# Autodesk Inventor assembly: full_layout_test
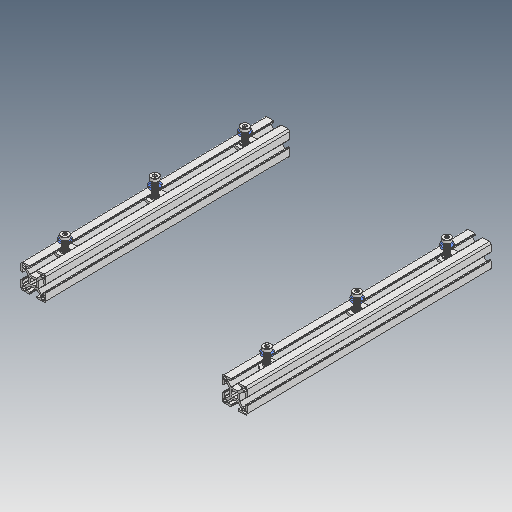
[picture p0: Inventor's stored thumbnail of the model, 512x512]
Saved by Autodesk Inventor 2025.4 (Build 294407020, 407B)
## iProperties
Created: 2026-09-08
Part Number: full_layout_test
Document SubType Name: Assembly
Designer: Aiden
Author: Aiden
## Documents named in this file (7)
- C:\Users\Aiden\Documents\GitHub\coldex-instrumentation\3d_models\mounting_hardware\dummy_parts\full_layout_test.iam
- C:\Users\Aiden\Documents\GitHub\coldex-instrumentation\3d_models\mounting_hardware\dummy_parts\acrylic_base.ipt
- C:\Users\Aiden\Documents\GitHub\coldex-instrumentation\3d_models\mounting_hardware\dummy_parts\acrylic_cover.ipt
- C:\Users\Aiden\Documents\GitHub\coldex-instrumentation\3d_models\mounting_hardware\McMaster\30mm_1ft_T-Slotted Framing.ipt
- C:\Users\Aiden\Documents\GitHub\coldex-instrumentation\3d_models\mounting_hardware\McMaster\30mm_teenut_T-Slotted Framing.ipt
- C:\Users\Aiden\Documents\GitHub\coldex-instrumentation\3d_models\mounting_hardware\McMaster\0.257in_innerD_Moisture-Resistant Cushioning Washer.ipt
- C:\Users\Aiden\Documents\GitHub\coldex-instrumentation\3d_models\mounting_hardware\McMaster\m6_18mm_18-8 Stainless Steel Low-Profile Socket Head Screws.ipt
## Components (22 placed, 6 different names)
1. acrylic_base:1 — Flush:1, Flush:2, Mate:1, Mate:2, Flush:3, Flush:4, Mate:9, Mate:10, Mate:11, Mate:12, Mate:13, Mate:14, Mate:21, Mate:22, Mate:23, Mate:24, Mate:25, Mate:26
2. acrylic_cover:1 — Flush:1, Flush:2
3. 30mm_1ft_T-Slotted Framing:1 — Mate:1, Flush:4, Mate:3, Mate:4, Mate:5, Tangent:2
4. 30mm_1ft_T-Slotted Framing:2 — Mate:2, Flush:3, Mate:6, Mate:7, Mate:8, Tangent:1
5. 30mm_teenut_T-Slotted Framing:1 — Mate:5, Mate:9
6. 30mm_teenut_T-Slotted Framing:2 — Mate:3, Mate:10
7. 30mm_teenut_T-Slotted Framing:3 — Mate:4, Mate:11, Tangent:2
8. 30mm_teenut_T-Slotted Framing:4 — Mate:7, Mate:13
9. 30mm_teenut_T-Slotted Framing:5 — Mate:6, Mate:14
10. 30mm_teenut_T-Slotted Framing:6 — Mate:8, Mate:12, Tangent:1
11. m6_18mm_18-8 Stainless Steel Low-Profile Socket Head Screws:1
12. m6_18mm_18-8 Stainless Steel Low-Profile Socket Head Screws:2
13. m6_18mm_18-8 Stainless Steel Low-Profile Socket Head Screws:3
14. m6_18mm_18-8 Stainless Steel Low-Profile Socket Head Screws:4
15. m6_18mm_18-8 Stainless Steel Low-Profile Socket Head Screws:5
16. m6_18mm_18-8 Stainless Steel Low-Profile Socket Head Screws:6
17. 0.257in_innerD_Moisture-Resistant Cushioning Washer:1 — Mate:22
18. 0.257in_innerD_Moisture-Resistant Cushioning Washer:2 — Mate:23
19. 0.257in_innerD_Moisture-Resistant Cushioning Washer:3 — Mate:24
20. 0.257in_innerD_Moisture-Resistant Cushioning Washer:4 — Mate:26
21. 0.257in_innerD_Moisture-Resistant Cushioning Washer:5 — Mate:25
22. 0.257in_innerD_Moisture-Resistant Cushioning Washer:6 — Mate:21
## Relationships (39: Mate 33, Flush 4, Tangent 2)
- Flush:1: acrylic_base:1 ↔ acrylic_cover:1
- Flush:2: acrylic_base:1 ↔ acrylic_cover:1
- Mate:1: acrylic_base:1 ↔ 30mm_1ft_T-Slotted Framing:1
- Mate:2: acrylic_base:1 ↔ 30mm_1ft_T-Slotted Framing:2
- Flush:3: acrylic_base:1 ↔ 30mm_1ft_T-Slotted Framing:2
- Flush:4: acrylic_base:1 ↔ 30mm_1ft_T-Slotted Framing:1
- Mate:3: 30mm_1ft_T-Slotted Framing:1 ↔ 30mm_teenut_T-Slotted Framing:2
- Mate:4: 30mm_1ft_T-Slotted Framing:1 ↔ 30mm_teenut_T-Slotted Framing:3
- Mate:5: 30mm_1ft_T-Slotted Framing:1 ↔ 30mm_teenut_T-Slotted Framing:1
- Mate:6: 30mm_1ft_T-Slotted Framing:2 ↔ 30mm_teenut_T-Slotted Framing:5
- Mate:7: 30mm_1ft_T-Slotted Framing:2 ↔ 30mm_teenut_T-Slotted Framing:4
- Mate:8: 30mm_1ft_T-Slotted Framing:2 ↔ 30mm_teenut_T-Slotted Framing:6
- Mate:9: acrylic_base:1 ↔ 30mm_teenut_T-Slotted Framing:1
- Mate:10: acrylic_base:1 ↔ 30mm_teenut_T-Slotted Framing:2
- Mate:11: acrylic_base:1 ↔ 30mm_teenut_T-Slotted Framing:3
- Mate:12: acrylic_base:1 ↔ 30mm_teenut_T-Slotted Framing:6
- Mate:13: acrylic_base:1 ↔ 30mm_teenut_T-Slotted Framing:4
- Mate:14: acrylic_base:1 ↔ 30mm_teenut_T-Slotted Framing:5
- Tangent:1: 30mm_1ft_T-Slotted Framing:2 ↔ 30mm_teenut_T-Slotted Framing:6
- Tangent:2: 30mm_1ft_T-Slotted Framing:1 ↔ 30mm_teenut_T-Slotted Framing:3
- [Mate]: acrylic_base:1 ↔ m6_18mm_18-8 Stainless Steel Low-Profile Socket Head Screws:1
- [Mate]: acrylic_base:1 ↔ m6_18mm_18-8 Stainless Steel Low-Profile Socket Head Screws:2
- [Mate]: acrylic_base:1 ↔ m6_18mm_18-8 Stainless Steel Low-Profile Socket Head Screws:3
- [Mate]: acrylic_base:1 ↔ m6_18mm_18-8 Stainless Steel Low-Profile Socket Head Screws:4
- [Mate]: acrylic_base:1 ↔ m6_18mm_18-8 Stainless Steel Low-Profile Socket Head Screws:5
- [Mate]: acrylic_base:1 ↔ m6_18mm_18-8 Stainless Steel Low-Profile Socket Head Screws:6
- Mate:21: acrylic_base:1 ↔ 0.257in_innerD_Moisture-Resistant Cushioning Washer:6
- Mate:22: acrylic_base:1 ↔ 0.257in_innerD_Moisture-Resistant Cushioning Washer:1
- Mate:23: acrylic_base:1 ↔ 0.257in_innerD_Moisture-Resistant Cushioning Washer:2
- Mate:24: acrylic_base:1 ↔ 0.257in_innerD_Moisture-Resistant Cushioning Washer:3
- Mate:25: acrylic_base:1 ↔ 0.257in_innerD_Moisture-Resistant Cushioning Washer:5
- Mate:26: acrylic_base:1 ↔ 0.257in_innerD_Moisture-Resistant Cushioning Washer:4
- [Mate]: m6_18mm_18-8 Stainless Steel Low-Profile Socket Head Screws:3 ↔ 0.257in_innerD_Moisture-Resistant Cushioning Washer:6
- [Mate]: m6_18mm_18-8 Stainless Steel Low-Profile Socket Head Screws:2 ↔ 0.257in_innerD_Moisture-Resistant Cushioning Washer:1
- [Mate]: m6_18mm_18-8 Stainless Steel Low-Profile Socket Head Screws:1 ↔ 0.257in_innerD_Moisture-Resistant Cushioning Washer:2
- [Mate]: m6_18mm_18-8 Stainless Steel Low-Profile Socket Head Screws:6 ↔ 0.257in_innerD_Moisture-Resistant Cushioning Washer:3
- [Mate]: m6_18mm_18-8 Stainless Steel Low-Profile Socket Head Screws:5 ↔ 0.257in_innerD_Moisture-Resistant Cushioning Washer:5
- [Mate]: m6_18mm_18-8 Stainless Steel Low-Profile Socket Head Screws:4 ↔ 0.257in_innerD_Moisture-Resistant Cushioning Washer:4
- [Mate]: m6_18mm_18-8 Stainless Steel Low-Profile Socket Head Screws:3 ↔ 0.257in_innerD_Moisture-Resistant Cushioning Washer:6
